# Autodesk Inventor assembly: Rear_Frame_Fixer_v4
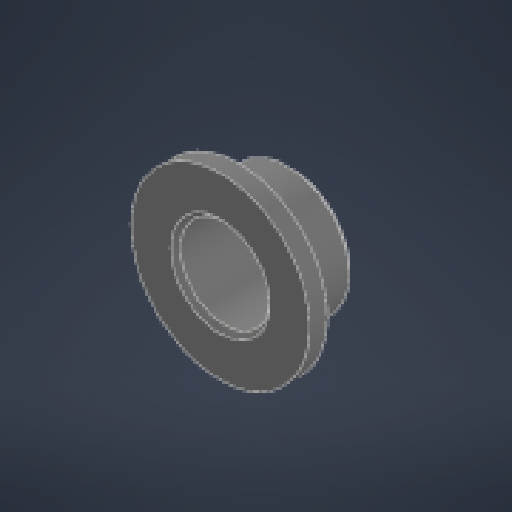
[picture p0: Inventor's stored thumbnail of the model, 512x512]
Saved by Autodesk Inventor 2024.3 (Build 283343000, 343)
## iProperties
Created: 2025-01-09
Part Number: Rear_Frame_Fixer_v4
Document SubType Name: Assembly
Designer: ASUS
Author: ASUS
## Documents named in this file (6)
- C:\Users\ASUS\Desktop\Anti_Backlash_Structure_OP\v4_Frame_2025\Rear_Frame_Fixer_v4.iam
- C:\Users\ASUS\Desktop\Anti_Backlash_Structure_OP\MISUMI\80F-0503.ipt
- C:\Users\ASUS\Desktop\Anti_Backlash_Structure_OP\MISUMI\C-WSSA12-4-2.ipt
- C:\Users\ASUS\Desktop\Anti_Backlash_Structure_OP\MISUMI\SLBNR4.ipt
- C:\Users\ASUS\Desktop\Anti_Backlash_Structure_OP\MISUMI\TT-0509-10.ipt
- C:\Users\ASUS\Desktop\Anti_Backlash_Structure_OP\v4_Frame_2025\ALI\Ali_d5-M4.ipt
## Components (5 placed, 5 different names)
1. 80F-0503:1 — 삽입:2, 삽입:3
2. C-WSSA12-4-2:1 — 삽입:1, 삽입:2
3. SLBNR4:1 — 삽입:1
4. TT-0509-10:1 — 삽입:3, 삽입:4
5. Ali_d5-M4:1 — 삽입:4
## Relationships (4: Insert 4)
- 삽입:1 [Insert] (1 mm): C-WSSA12-4-2:1 ↔ SLBNR4:1
- 삽입:2 [Insert]: 80F-0503:1 ↔ C-WSSA12-4-2:1
- 삽입:3 [Insert]: 80F-0503:1 ↔ TT-0509-10:1
- 삽입:4 [Insert]: TT-0509-10:1 ↔ Ali_d5-M4:1
